# Autodesk Inventor assembly: 545588
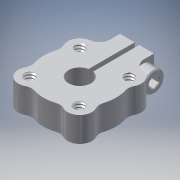
[picture p0: Inventor's stored thumbnail of the model, 180x180]
Saved by Autodesk Inventor 2016 SP2 (Build 200236200, 236)
## iProperties
Created: 2016-08-18
Part Number: 545588
Description: Face Tapped Clamping Hub (0.77in)
Document SubType Name: Assembly
Designer: 589013
Mass: 7.88454 g
Surface Area: 26.2506 cm^2
Volume: 2.9202 cm^3
Density: 2.7 g/cm^3
Sending System: SolidWorks 2014
Preprocessor: SwSTEP 2.0
Title: 545588 assembly.STEP
Revision Number: ANY
## Documents named in this file (3)
- E:\GrabCAD\Power Hawks CAD\ServoCity Resources\Hubs\FaceTappedClampingHub(0.77in)-1111-2017.iam
- E:\GrabCAD\Power Hawks CAD\ServoCity Resources\Hubs\Face Tapped Clamping Hub\FaceTappedClampingHub(0.77in)(Hub)-1111-2017.ipt
- E:\GrabCAD\Power Hawks CAD\ServoCity Resources\Hubs\Face Tapped Clamping Hub\FaceTappedClampingHub(0.77in)(Screw)-1111-2017.ipt
## Components (2 placed, 2 different names)
1. 545588_1 — Insert:1
2. 632110_90128A121_2 — Insert:1
## Relationships (1: Insert 1)
- Insert:1: 545588_1 ↔ 632110_90128A121_2
